# Autodesk Inventor assembly: Stamp Assembly
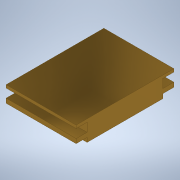
[picture p0: Inventor's stored thumbnail of the model, 180x180]
Saved by Autodesk Inventor 2022 (Build 260153000, 153)
## iProperties
Created: 2021-01-06
Part Number: Stamp Assembly
Document SubType Name: Assembly
Designer: caleb
Author: caleb
## Documents named in this file (3)
- C:\Users\Caleb\Desktop\nebraska-silicon-lab\Hardware\ETL\Module Assembly\Glue Stamp - V2\Stamp Assembly - V2.iam
- C:\Users\Caleb\Desktop\nebraska-silicon-lab\Hardware\ETL\Module Assembly\Glue Stamp - V2\Rubber Stamp - V2.ipt
- C:\Users\Caleb\Desktop\nebraska-silicon-lab\Hardware\ETL\Module Assembly\Glue Stamp - V2\Stamp Body - V2.ipt
## Components (2 placed, 2 different names)
1. Rubber Stamp - V2:1 — Mate:1, Angle:1, Flush:1, Flush:2
2. Stamp Body - V2:1 — Mate:1, Angle:1, Flush:1, Flush:2
## Relationships (4: Flush 2, Mate 1, Angle 1)
- Mate:1: Rubber Stamp - V2:1 ↔ Stamp Body - V2:1
- Angle:1 (0 deg): Rubber Stamp - V2:1 ↔ Stamp Body - V2:1
- Flush:1 (1 mm): Rubber Stamp - V2:1 ↔ Stamp Body - V2:1
- Flush:2 (1 mm): Rubber Stamp - V2:1 ↔ Stamp Body - V2:1
